# Autodesk Inventor assembly: car_2
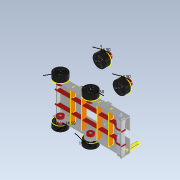
[picture p0: Inventor's stored thumbnail of the model, 180x180]
Saved by Autodesk Inventor 2022 (Build 260153000, 153)
## iProperties
Created: 2023-04-28
Part Number: car_2
Document SubType Name: Assembly
Designer: Johnny Jou
Author: Johnny Jou
## Documents named in this file (15)
- C:\Users\Johnny Jou\Documents\GitHub\Areo_Rider_Cabin\car\car_2.iam
- C:\Users\Johnny Jou\Documents\GitHub\Areo_Rider_Cabin\car\chassis_1_1_3.ipt
- C:\Users\Johnny Jou\Documents\GitHub\Areo_Rider_Cabin\car\外抓檔\25GA370.ipt
- C:\Users\Johnny Jou\Documents\GitHub\Areo_Rider_Cabin\car\chassis_1_5.ipt
- C:\Users\Johnny Jou\Documents\GitHub\Areo_Rider_Cabin\car\chassis_1_6.ipt
- C:\Users\Johnny Jou\Documents\GitHub\Areo_Rider_Cabin\car\plate_2.ipt
- C:\Users\Johnny Jou\Documents\GitHub\Areo_Rider_Cabin\car\bracket.ipt
- C:\Users\Johnny Jou\Documents\GitHub\Areo_Rider_Cabin\car\wheel.ipt
- C:\Users\Johnny Jou\Documents\GitHub\Areo_Rider_Cabin\car\chassis_1_7.ipt
- C:\Users\Johnny Jou\Documents\GitHub\Areo_Rider_Cabin\car\Coupling_0504.ipt
- C:\Users\Johnny Jou\Documents\GitHub\Areo_Rider_Cabin\car\2GT_36T.ipt
- C:\Users\Johnny Jou\Documents\GitHub\Areo_Rider_Cabin\car\2GT_60T.ipt
- C:\Users\Johnny Jou\Documents\GitHub\Areo_Rider_Cabin\car\axle 4_20.ipt
- C:\Users\Johnny Jou\Documents\GitHub\Areo_Rider_Cabin\car\bearing.ipt
- C:\Users\Johnny Jou\Documents\GitHub\Areo_Rider_Cabin\car\wheel_base_cover.ipt
## Components (57 placed, 14 different names)
1. 25GA370:1 — 貼合:7, 貼合:9
2. 25GA370:2 — 貼合:7, 貼合:8, 貼合:49
3. chassis_1_5:1 — 貼合:9, 齊平:5, 齊平:10, 齊平:11, 齊平:12, 齊平:13, 貼合:13, 貼合:14, 貼合:42, 貼合:43, 貼合:51
4. chassis_1_5:2 — 貼合:8, 齊平:5, 貼合:15, 貼合:16, 貼合:17, 貼合:18, 貼合:19, 貼合:20
5. chassis_1_6:1 — 齊平:7, 齊平:8, 齊平:9, 齊平:13, 貼合:13, 貼合:14
6. chassis_1_6:2 — 齊平:8, 齊平:10, 貼合:17, 貼合:18, 貼合:42, 貼合:43, 齊平:14, 貼合:44, 貼合:45, 齊平:15
7. chassis_1_6:3 — 齊平:9, 齊平:11, 貼合:19, 貼合:20
8. chassis_1_6:4 — 齊平:7, 齊平:12, 貼合:15, 貼合:16
9. plate_2:1 — 貼合:38, 貼合:40, 貼合:41, 貼合:50, 齊平:18, 齊平:19
10. bracket:7 — 貼合:38, 貼合:40
11. bracket:8 — 貼合:41
12. chassis_1_1_3:1 — 齊平:14, 貼合:44, 貼合:45, 貼合:46, 貼合:47, 貼合:48, 貼合:49, 齊平:16, 齊平:17, 齊平:18, 貼合:108, 貼合:110, 貼合:111, 貼合:154, 貼合:155
13. chassis_1_1_3:2 — 齊平:15, 齊平:16, 齊平:17, 貼合:50, 齊平:19, 貼合:52, 貼合:53, 貼合:54, 貼合:55, 貼合:56, 貼合:57, 貼合:109, 貼合:156, 貼合:157
14. wheel:1 — 貼合:58, 貼合:59
15. chassis_1_7:1 — 貼合:51, 貼合:52, 貼合:53
16. chassis_1_7:2 — 貼合:54, 貼合:55, 貼合:56, 貼合:57
17. Coupling_0504:1 — 貼合:58, 貼合:59, 貼合:60, 貼合:61, 貼合:62, 貼合:63, 貼合:64, 貼合:66
18. 2GT_36T:1 — 貼合:60, 貼合:61, 貼合:62, 貼合:65
19. 2GT_60T:1 — 齊平:25, 貼合:124, 貼合:125, 貼合:127
20. 2GT_36T:2 — 貼合:63, 貼合:64, 貼合:65, 貼合:70
21. axle 4_20:1 — 貼合:66, 貼合:69, 齊平:20
22. 軸承 GB/T 292-2007 類型 IN - 退回 B724 C:1 — 貼合:67, 貼合:68, 貼合:69, 齊平:20
23. wheel_base_cover:1 — 貼合:67, 貼合:68, 貼合:70
24. wheel:2
25. Coupling_0504:2
26. 2GT_36T:3
27. 2GT_36T:4
28. axle 4_20:2
29. 軸承 GB/T 292-2007 類型 IN - 退回 B724 C:2
30. wheel_base_cover:2 — 貼合:108, 貼合:109
31. wheel:3
32. Coupling_0504:4
33. 2GT_36T:7
34. 2GT_36T:8
35. axle 4_20:4
36. 軸承 GB/T 292-2007 類型 IN - 退回 B724 C:4
37. wheel_base_cover:4 — 貼合:110, 貼合:111
38. wheel:4
39. Coupling_0504:5 — 貼合:126, 貼合:127, 貼合:128
40. axle 4_20:5
41. 軸承 GB/T 292-2007 類型 IN - 退回 B724 C:5
42. wheel_base_cover:5 — 貼合:129, 貼合:156, 貼合:157
43. 2GT_60T:2 — 齊平:25, 貼合:124, 貼合:125, 貼合:126, 貼合:128, 貼合:129
44. 2GT_60T:3
45. wheel:5
46. Coupling_0504:6
47. axle 4_20:6
48. 軸承 GB/T 292-2007 類型 IN - 退回 B724 C:6
49. wheel_base_cover:6
50. 2GT_60T:4
51. 2GT_60T:5
52. wheel:6
53. Coupling_0504:7
54. axle 4_20:7
55. 軸承 GB/T 292-2007 類型 IN - 退回 B724 C:7
56. wheel_base_cover:7 — 貼合:154, 貼合:155
57. 2GT_60T:6
## Relationships (139: Mate 116, Flush 23)
- 貼合:7 [Mate] (20 mm): 25GA370:1 ↔ 25GA370:2
- 貼合:8 [Mate]: 25GA370:2 ↔ chassis_1_5:2
- 貼合:9 [Mate]: 25GA370:1 ↔ chassis_1_5:1
- 齊平:5 [Flush]: chassis_1_5:1 ↔ chassis_1_5:2
- 齊平:7 [Flush]: chassis_1_6:1 ↔ chassis_1_6:4
- 齊平:8 [Flush]: chassis_1_6:1 ↔ chassis_1_6:2
- 齊平:9 [Flush]: chassis_1_6:1 ↔ chassis_1_6:3
- 齊平:10 [Flush]: chassis_1_5:1 ↔ chassis_1_6:2
- 齊平:11 [Flush]: chassis_1_5:1 ↔ chassis_1_6:3
- 齊平:12 [Flush]: chassis_1_5:1 ↔ chassis_1_6:4
- 齊平:13 [Flush]: chassis_1_5:1 ↔ chassis_1_6:1
- 貼合:13 [Mate]: chassis_1_5:1 ↔ chassis_1_6:1
- 貼合:14 [Mate]: chassis_1_5:1 ↔ chassis_1_6:1
- 貼合:15 [Mate]: chassis_1_5:2 ↔ chassis_1_6:4
- 貼合:16 [Mate]: chassis_1_5:2 ↔ chassis_1_6:4
- 貼合:17 [Mate]: chassis_1_5:2 ↔ chassis_1_6:2
- 貼合:18 [Mate]: chassis_1_5:2 ↔ chassis_1_6:2
- 貼合:19 [Mate]: chassis_1_5:2 ↔ chassis_1_6:3
- 貼合:20 [Mate]: chassis_1_5:2 ↔ chassis_1_6:3
- [Mate]: bracket:7 ↔ bracket:8
- [Mate]: bracket:7 ↔ bracket:8
- [Mate]: bracket:7 ↔ bracket:8
- 貼合:38 [Mate]: plate_2:1 ↔ bracket:7
- 貼合:40 [Mate]: plate_2:1 ↔ bracket:7
- 貼合:41 [Mate]: plate_2:1 ↔ bracket:8
- 貼合:42 [Mate]: chassis_1_5:1 ↔ chassis_1_6:2
- 貼合:43 [Mate]: chassis_1_5:1 ↔ chassis_1_6:2
- 齊平:14 [Flush]: chassis_1_6:2 ↔ chassis_1_1_3:1
- 貼合:44 [Mate]: chassis_1_6:2 ↔ chassis_1_1_3:1
- 貼合:45 [Mate]: chassis_1_6:2 ↔ chassis_1_1_3:1
- 貼合:46 [Mate]: chassis_1_1_3:1
- 貼合:47 [Mate]: chassis_1_1_3:1
- 貼合:48 [Mate]: chassis_1_1_3:1
- 貼合:49 [Mate]: 25GA370:2 ↔ chassis_1_1_3:1
- 齊平:15 [Flush]: chassis_1_6:2 ↔ chassis_1_1_3:2
- 齊平:16 [Flush]: chassis_1_1_3:1 ↔ chassis_1_1_3:2
- 齊平:17 [Flush]: chassis_1_1_3:1 ↔ chassis_1_1_3:2
- 貼合:50 [Mate]: plate_2:1 ↔ chassis_1_1_3:2
- 齊平:18 [Flush]: plate_2:1 ↔ chassis_1_1_3:1
- 齊平:19 [Flush]: plate_2:1 ↔ chassis_1_1_3:2
- 貼合:51 [Mate]: chassis_1_5:1 ↔ chassis_1_7:1
- 貼合:52 [Mate]: chassis_1_1_3:2 ↔ chassis_1_7:1
- 貼合:53 [Mate]: chassis_1_1_3:2 ↔ chassis_1_7:1
- 貼合:54 [Mate]: chassis_1_1_3:2 ↔ chassis_1_7:2
- 貼合:55 [Mate]: chassis_1_1_3:2 ↔ chassis_1_7:2
- 貼合:56 [Mate]: chassis_1_1_3:2 ↔ chassis_1_7:2
- 貼合:57 [Mate]: chassis_1_1_3:2 ↔ chassis_1_7:2
- 貼合:58 [Mate]: wheel:1 ↔ Coupling_0504:1
- 貼合:59 [Mate]: wheel:1 ↔ Coupling_0504:1
- 貼合:60 [Mate]: Coupling_0504:1 ↔ 2GT_36T:1
- 貼合:61 [Mate]: Coupling_0504:1 ↔ 2GT_36T:1
- 貼合:62 [Mate]: Coupling_0504:1 ↔ 2GT_36T:1
- 貼合:63 [Mate]: Coupling_0504:1 ↔ 2GT_36T:2
- 貼合:64 [Mate]: Coupling_0504:1 ↔ 2GT_36T:2
- 貼合:65 [Mate]: 2GT_36T:1 ↔ 2GT_36T:2
- 貼合:66 [Mate]: Coupling_0504:1 ↔ axle 4_20:1
- 貼合:67 [Mate]: 軸承 GB/T 292-2007 類型 IN - 退回 B724 C:1 ↔ wheel_base_cover:1
- 貼合:68 [Mate]: 軸承 GB/T 292-2007 類型 IN - 退回 B724 C:1 ↔ wheel_base_cover:1
- 貼合:69 [Mate]: axle 4_20:1 ↔ 軸承 GB/T 292-2007 類型 IN - 退回 B724 C:1
- 齊平:20 [Flush]: axle 4_20:1 ↔ 軸承 GB/T 292-2007 類型 IN - 退回 B724 C:1
- 貼合:70 [Mate] (5 mm): 2GT_36T:2 ↔ wheel_base_cover:1
- [Mate]: wheel:2 ↔ Coupling_0504:2
- [Mate]: wheel:2 ↔ Coupling_0504:2
- [Mate]: Coupling_0504:2 ↔ 2GT_36T:3
- [Mate]: Coupling_0504:2 ↔ 2GT_36T:3
- [Mate]: Coupling_0504:2 ↔ 2GT_36T:3
- [Mate]: Coupling_0504:2 ↔ 2GT_36T:4
- [Mate]: Coupling_0504:2 ↔ 2GT_36T:4
- [Mate]: 2GT_36T:3 ↔ 2GT_36T:4
- [Mate]: Coupling_0504:2 ↔ axle 4_20:2
- [Mate]: 軸承 GB/T 292-2007 類型 IN - 退回 B724 C:2 ↔ wheel_base_cover:2
- [Mate]: 軸承 GB/T 292-2007 類型 IN - 退回 B724 C:2 ↔ wheel_base_cover:2
- [Mate]: axle 4_20:2 ↔ 軸承 GB/T 292-2007 類型 IN - 退回 B724 C:2
- [Flush]: axle 4_20:2 ↔ 軸承 GB/T 292-2007 類型 IN - 退回 B724 C:2
- [Mate] (5 mm): 2GT_36T:4 ↔ wheel_base_cover:2
- [Mate]: wheel:3 ↔ Coupling_0504:4
- [Mate]: wheel:3 ↔ Coupling_0504:4
- [Mate]: Coupling_0504:4 ↔ 2GT_36T:7
- [Mate]: Coupling_0504:4 ↔ 2GT_36T:7
- [Mate]: Coupling_0504:4 ↔ 2GT_36T:7
- [Mate]: Coupling_0504:4 ↔ 2GT_36T:8
- [Mate]: Coupling_0504:4 ↔ 2GT_36T:8
- [Mate]: 2GT_36T:7 ↔ 2GT_36T:8
- [Mate]: Coupling_0504:4 ↔ axle 4_20:4
- [Mate]: 軸承 GB/T 292-2007 類型 IN - 退回 B724 C:4 ↔ wheel_base_cover:4
- [Mate]: 軸承 GB/T 292-2007 類型 IN - 退回 B724 C:4 ↔ wheel_base_cover:4
- [Mate]: axle 4_20:4 ↔ 軸承 GB/T 292-2007 類型 IN - 退回 B724 C:4
- [Flush]: axle 4_20:4 ↔ 軸承 GB/T 292-2007 類型 IN - 退回 B724 C:4
- [Mate] (5 mm): 2GT_36T:8 ↔ wheel_base_cover:4
- 貼合:108 [Mate]: chassis_1_1_3:1 ↔ wheel_base_cover:2
- 貼合:109 [Mate]: chassis_1_1_3:2 ↔ wheel_base_cover:2
- 貼合:110 [Mate]: chassis_1_1_3:1 ↔ wheel_base_cover:4
- 貼合:111 [Mate]: chassis_1_1_3:1 ↔ wheel_base_cover:4
- [Mate]: wheel:4 ↔ Coupling_0504:5
- [Mate]: wheel:4 ↔ Coupling_0504:5
- [Mate]: Coupling_0504:5 ↔ axle 4_20:5
- [Mate]: 軸承 GB/T 292-2007 類型 IN - 退回 B724 C:5 ↔ wheel_base_cover:5
- [Mate]: 軸承 GB/T 292-2007 類型 IN - 退回 B724 C:5 ↔ wheel_base_cover:5
- [Mate]: axle 4_20:5 ↔ 軸承 GB/T 292-2007 類型 IN - 退回 B724 C:5
- [Flush]: axle 4_20:5 ↔ 軸承 GB/T 292-2007 類型 IN - 退回 B724 C:5
- 齊平:25 [Flush]: 2GT_60T:1 ↔ 2GT_60T:2
- 貼合:124 [Mate]: 2GT_60T:1 ↔ 2GT_60T:2
- 貼合:125 [Mate]: 2GT_60T:1 ↔ 2GT_60T:2
- 貼合:126 [Mate]: Coupling_0504:5 ↔ 2GT_60T:2
- 貼合:127 [Mate]: 2GT_60T:1 ↔ Coupling_0504:5
- 貼合:128 [Mate]: Coupling_0504:5 ↔ 2GT_60T:2
- 貼合:129 [Mate] (5 mm): wheel_base_cover:5 ↔ 2GT_60T:2
- [Mate]: wheel:5 ↔ Coupling_0504:6
- [Mate]: wheel:5 ↔ Coupling_0504:6
- [Mate]: Coupling_0504:6 ↔ axle 4_20:6
- [Mate]: 軸承 GB/T 292-2007 類型 IN - 退回 B724 C:6 ↔ wheel_base_cover:6
- [Mate]: 軸承 GB/T 292-2007 類型 IN - 退回 B724 C:6 ↔ wheel_base_cover:6
- [Mate]: axle 4_20:6 ↔ 軸承 GB/T 292-2007 類型 IN - 退回 B724 C:6
- [Flush]: axle 4_20:6 ↔ 軸承 GB/T 292-2007 類型 IN - 退回 B724 C:6
- [Flush]: 2GT_60T:3 ↔ 2GT_60T:4
- [Mate]: 2GT_60T:3 ↔ 2GT_60T:4
- [Mate]: 2GT_60T:3 ↔ 2GT_60T:4
- [Mate]: Coupling_0504:6 ↔ 2GT_60T:4
- [Mate]: 2GT_60T:3 ↔ Coupling_0504:6
- [Mate]: Coupling_0504:6 ↔ 2GT_60T:4
- [Mate] (5 mm): wheel_base_cover:6 ↔ 2GT_60T:4
- [Mate]: wheel:6 ↔ Coupling_0504:7
- [Mate]: wheel:6 ↔ Coupling_0504:7
- [Mate]: Coupling_0504:7 ↔ axle 4_20:7
- [Mate]: 軸承 GB/T 292-2007 類型 IN - 退回 B724 C:7 ↔ wheel_base_cover:7
- [Mate]: 軸承 GB/T 292-2007 類型 IN - 退回 B724 C:7 ↔ wheel_base_cover:7
- [Mate]: axle 4_20:7 ↔ 軸承 GB/T 292-2007 類型 IN - 退回 B724 C:7
- [Flush]: axle 4_20:7 ↔ 軸承 GB/T 292-2007 類型 IN - 退回 B724 C:7
- [Flush]: 2GT_60T:5 ↔ 2GT_60T:6
- [Mate]: 2GT_60T:5 ↔ 2GT_60T:6
- [Mate]: 2GT_60T:5 ↔ 2GT_60T:6
- [Mate]: Coupling_0504:7 ↔ 2GT_60T:6
- [Mate]: 2GT_60T:5 ↔ Coupling_0504:7
- [Mate]: Coupling_0504:7 ↔ 2GT_60T:6
- [Mate] (5 mm): wheel_base_cover:7 ↔ 2GT_60T:6
- 貼合:154 [Mate]: chassis_1_1_3:1 ↔ wheel_base_cover:7
- 貼合:155 [Mate]: chassis_1_1_3:1 ↔ wheel_base_cover:7
- 貼合:156 [Mate]: chassis_1_1_3:2 ↔ wheel_base_cover:5
- 貼合:157 [Mate]: chassis_1_1_3:2 ↔ wheel_base_cover:5
## Named parameters: d54_d45 = 0 mm, d55_d46 = 0 mm, d56_d47 = 0 mm, d112_d98 = 0 mm, d113_d99 = 0 mm, d114_d100 = 0 mm, d115_d101 = 0 mm, d116_d102 = 0 mm, d117_d103 = 0 mm, d118_d104 = 0 mm, d119_d105 = 0 mm, d120_d106 = 0 mm, d121_d107 = 0 mm, d122_d108 = 0 mm, d123_d109 = 0 mm, d124_d110 = 0 mm, d125_d111 = 5 mm, d138_d98 = 0 mm, d139_d99 = 0 mm, d140_d100 = 0 mm, d141_d101 = 0 mm, d142_d102 = 0 mm, d143_d103 = 0 mm, d144_d104 = 0 mm, d145_d105 = 0 mm, d146_d106 = 0 mm, d147_d107 = 0 mm, d148_d108 = 0 mm, d149_d109 = 0 mm, d150_d110 = 0 mm, d151_d111 = 5 mm, d156_d98 = 0 mm, d157_d99 = 0 mm, d164_d106 = 0 mm, d165_d107 = 0 mm, d166_d108 = 0 mm, d167_d109 = 0 mm, d168_d110 = 0 mm, d177_d170 = 0 mm, d178_d171 = 0 mm, d179_d172 = 0 mm, d180_d173 = 0 mm, d181_d174 = 0 mm, d182_d175 = 0 mm, d183_d176 = 5 mm, d184_d156_d98 = 0 mm, d185_d157_d99 = 0 mm, d186_d164_d106 = 0 mm, d187_d165_d107 = 0 mm, d188_d166_d108 = 0 mm, d189_d167_d109 = 0 mm, d190_d168_d110 = 0 mm, d191_d170 = 0 mm, d192_d171 = 0 mm, d193_d172 = 0 mm, d194_d173 = 0 mm, d195_d174 = 0 mm, d196_d175 = 0 mm, d197_d176 = 5 mm, d198_d156_d98 = 0 mm, d199_d157_d99 = 0 mm, d200_d164_d106 = 0 mm, d201_d165_d107 = 0 mm, d202_d166_d108 = 0 mm, d203_d167_d109 = 0 mm, d204_d168_d110 = 0 mm
